# Autodesk Inventor assembly: marco
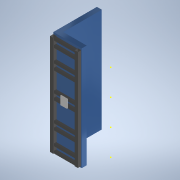
[picture p0: Inventor's stored thumbnail of the model, 180x180]
Saved by Autodesk Inventor 2021.2 (Build 252289000, 289)
## iProperties
Created: 2021-04-11
Part Number: marco
Document SubType Name: Assembly
Designer: equip
Mass: 525959 g
Surface Area: 133006 cm^2
Volume: 315655 cm^3
Density: 1.66625 g/cm^3
_SolveAssemblyDoc: Frame Generator Solve Assembly
_Version: 25.0.0
Author: equip
## Documents named in this file (5)
- C:\Users\equip\Documents\AAA Nacho Mecatrónica\Nacho Sexto Semestre MT\Diseño Mecatrónico\inventor proyecto\marco.iam
- C:\Users\equip\Documents\AAA Nacho Mecatrónica\Nacho Sexto Semestre MT\Diseño Mecatrónico\inventor proyecto\Marco central.ipt
- C:\Users\equip\Documents\AAA Nacho Mecatrónica\Nacho Sexto Semestre MT\Diseño Mecatrónico\inventor proyecto\marco\Frame\Frame 1618182230761.iam
- C:\Users\equip\Documents\AAA Nacho Mecatrónica\Nacho Sexto Semestre MT\Diseño Mecatrónico\inventor proyecto\placa centro.ipt
- C:\Users\equip\Documents\AAA Nacho Mecatrónica\Nacho Sexto Semestre MT\Diseño Mecatrónico\inventor proyecto\Silla del marco.ipt
## Components (7 placed, 4 different names)
1. Marco central:1
2. Frame 1618182230761:1 [sub-assembly] — Coincidencia:1, Nivelación:1, Coincidencia:2, Nivelación:2, Coincidencia:3, Nivelación:3, Nivelación:4, Coincidencia:4, Nivelación:5, Coincidencia:5, Nivelación:8, Coincidencia:6
3. placa centro:1 — Coincidencia:1, Nivelación:1, Coincidencia:2
4. Silla del marco:1 — Nivelación:2, Coincidencia:3, Nivelación:3, Coincidencia:7
5. Silla del marco:2 — Nivelación:4, Coincidencia:4, Coincidencia:7, Coincidencia:8
6. Silla del marco:3 — Nivelación:5, Coincidencia:5, Coincidencia:8, Coincidencia:9
7. Silla del marco:4 — Nivelación:8, Coincidencia:6, Coincidencia:9
## Relationships (15: Mate 9, Flush 6)
- Coincidencia:1 [Mate]: Frame 1618182230761:1 ↔ placa centro:1
- Nivelación:1 [Flush]: Frame 1618182230761:1 ↔ placa centro:1
- Coincidencia:2 [Mate] (150 mm): Frame 1618182230761:1 ↔ placa centro:1
- Nivelación:2 [Flush]: Frame 1618182230761:1 ↔ Silla del marco:1
- Coincidencia:3 [Mate]: Frame 1618182230761:1 ↔ Silla del marco:1
- Nivelación:3 [Flush] (-37.5 mm): Frame 1618182230761:1 ↔ Silla del marco:1
- Nivelación:4 [Flush]: Frame 1618182230761:1 ↔ Silla del marco:2
- Coincidencia:4 [Mate]: Frame 1618182230761:1 ↔ Silla del marco:2
- Nivelación:5 [Flush]: Frame 1618182230761:1 ↔ Silla del marco:3
- Coincidencia:5 [Mate]: Frame 1618182230761:1 ↔ Silla del marco:3
- Nivelación:8 [Flush]: Frame 1618182230761:1 ↔ Silla del marco:4
- Coincidencia:6 [Mate]: Frame 1618182230761:1 ↔ Silla del marco:4
- Coincidencia:7 [Mate]: Silla del marco:1 ↔ Silla del marco:2
- Coincidencia:8 [Mate]: Silla del marco:2 ↔ Silla del marco:3
- Coincidencia:9 [Mate]: Silla del marco:3 ↔ Silla del marco:4
## Named parameters: sa_0 = 470880, sa_1 = 470880, sa_2 = 470880, sa_3 = 470880, sa_4 = 1000, sa_5 = 1e+06, sa_6 = 1e+06
note: some values were not read from the file. Shown as the stored number, unit unknown: "sa_0", "sa_1", "sa_2", "sa_3", "sa_4", "sa_5", "sa_6".
